# Autodesk Inventor assembly: 膝_6_1
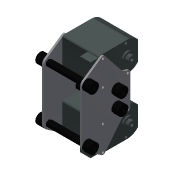
[picture p0: Inventor's stored thumbnail of the model, 180x180]
Saved by Autodesk Inventor 2016 (Build 200138000, 138)
## iProperties
Created: 2016-08-23
Part Number: 膝_6_1
Material: 一般
Document SubType Name: Assembly
Designer: hiro
Mass: 259.679 g
Surface Area: 513.454 cm^2
Volume: 137.54 cm^3
Density: 1.88802 g/cm^3
Author: hiro
## Documents named in this file (11)
- C:\Users\haya\Desktop\OpenPlatform\下半身_160823\膝\膝_6_1_MIR.iam
- C:\Users\haya\Desktop\OpenPlatform\既製品\B3M11xx.ipt
- B3M11xx.ipt
- C:\Users\haya\Desktop\OpenPlatform\下半身_160823\膝\膝_メインフレーム_6_1.ipt
- C:\Users\haya\Desktop\OpenPlatform\下半身_160823\膝\膝_サブフレーム_6_4.ipt
- C:\Users\haya\Desktop\OpenPlatform\既製品\新規購入\AMP-340E.ipt
- C:\Users\haya\Desktop\OpenPlatform\既製品\新規購入\BRU-306_5.ipt
- C:\Users\haya\Desktop\OpenPlatform\既製品\新規購入\D3040-7815B.ipt
- C:\Users\haya\Desktop\OpenPlatform\既製品\新規購入\D3040-7115B.ipt
- C:\Users\haya\Desktop\OpenPlatform\既製品\新規購入\LL-7211-08.ipt
- C:\Users\haya\Desktop\OpenPlatform\既製品\新規購入\LL-7211-10.ipt
## Components (40 placed, 9 different names)
1. B3M11xx:1 — メイト:1, メイト:2, フラッシュ:1, 挿入:1, 挿入:2, 挿入:3, 挿入:7, 挿入:10, 挿入:11
2. 膝_メインフレーム_6_1:1 — 挿入:1, 挿入:2, 挿入:3, 挿入:4, 挿入:5, 挿入:6, 挿入:34, 挿入:35, 挿入:36, 挿入:37, 挿入:38, 挿入:39, 角度:1, 角度:2, 角度:3, 角度:4, 挿入:44, 挿入:45, 挿入:58, 挿入:59, 挿入:60, 挿入:61
3. B3M11xx:2 — 挿入:4, 挿入:5, 挿入:6, 挿入:8, 挿入:9, 挿入:12
4. 膝_メインフレーム_6_1:2 — 挿入:7, 挿入:8, 挿入:9, 挿入:10, 挿入:11, 挿入:12, 挿入:40, 挿入:41, 挿入:42, 挿入:43, メイト:3, メイト:4, メイト:5, メイト:6, メイト:7, メイト:8, メイト:9, メイト:10
5. 膝_サブフレーム_6_4:1 — 挿入:34
6. 膝_サブフレーム_6_4:2 — 挿入:35
7. AMP-340E:1 — 挿入:36, 挿入:43, 角度:1
8. AMP-340E:2 — 挿入:37, 挿入:42, 角度:4
9. AMP-340E:3 — 挿入:38, 挿入:40, 角度:2
10. AMP-340E:4 — 挿入:39, 挿入:41, 角度:3
11. 膝_サブフレーム_6_4:3 — メイト:6, メイト:9, 挿入:56
12. 膝_サブフレーム_6_4:4 — メイト:5, メイト:10, 挿入:54
13. 膝_サブフレーム_6_4:5 — メイト:3, メイト:4, 挿入:55
14. 膝_サブフレーム_6_4:6 — メイト:7, メイト:8, 挿入:57
15. 膝_サブフレーム_6_4:7 — 挿入:44
16. 膝_サブフレーム_6_4:8 — 挿入:45
17. BRU-306_5:1 — 挿入:60, 挿入:93
18. BRU-306_5:2 — 挿入:61, 挿入:92
19. BRU-306_5:3 — 挿入:57, 挿入:90
20. BRU-306_5:4 — 挿入:54, 挿入:88
21. BRU-306_5:5 — 挿入:59, 挿入:91
22. BRU-306_5:6 — 挿入:58, 挿入:87
23. BRU-306_5:7 — 挿入:56, 挿入:89
24. BRU-306_5:8 — 挿入:55, 挿入:86
25. D3040-7815B:1 — 挿入:79, 挿入:90
26. D3040-7815B:2 — 挿入:80, 挿入:88
27. D3040-7815B:3 — 挿入:78, 挿入:86
28. D3040-7815B:4 — 挿入:81, 挿入:89
29. D3040-7115B:1 — 挿入:85, 挿入:91
30. D3040-7115B:2 — 挿入:84, 挿入:92
31. D3040-7115B:3 — 挿入:83, 挿入:93
32. D3040-7115B:4 — 挿入:82, 挿入:87
33. LL-7211-08:1 — 挿入:81
34. LL-7211-08:2 — 挿入:79
35. LL-7211-08:3 — 挿入:80
36. LL-7211-08:4 — 挿入:78
37. LL-7211-10:1 — 挿入:85
38. LL-7211-10:2 — 挿入:82
39. LL-7211-10:3 — 挿入:83
40. LL-7211-10:4 — 挿入:84
## Relationships (63: Insert 48, Mate 10, Angle 4, Flush 1)
- メイト:1 [Mate] (-19.75 mm): B3M11xx:1
- メイト:2 [Mate] (-25.75 mm): B3M11xx:1
- フラッシュ:1 [Flush] (38 mm): B3M11xx:1
- 挿入:1 [Insert]: B3M11xx:1 ↔ 膝_メインフレーム_6_1:1
- 挿入:2 [Insert]: B3M11xx:1 ↔ 膝_メインフレーム_6_1:1
- 挿入:3 [Insert]: B3M11xx:1 ↔ 膝_メインフレーム_6_1:1
- 挿入:4 [Insert]: 膝_メインフレーム_6_1:1 ↔ B3M11xx:2
- 挿入:5 [Insert]: 膝_メインフレーム_6_1:1 ↔ B3M11xx:2
- 挿入:6 [Insert]: 膝_メインフレーム_6_1:1 ↔ B3M11xx:2
- 挿入:7 [Insert]: B3M11xx:1 ↔ 膝_メインフレーム_6_1:2
- 挿入:8 [Insert]: B3M11xx:2 ↔ 膝_メインフレーム_6_1:2
- 挿入:9 [Insert]: B3M11xx:2 ↔ 膝_メインフレーム_6_1:2
- 挿入:10 [Insert]: B3M11xx:1 ↔ 膝_メインフレーム_6_1:2
- 挿入:11 [Insert]: B3M11xx:1 ↔ 膝_メインフレーム_6_1:2
- 挿入:12 [Insert]: B3M11xx:2 ↔ 膝_メインフレーム_6_1:2
- 挿入:34 [Insert]: 膝_メインフレーム_6_1:1 ↔ 膝_サブフレーム_6_4:1
- 挿入:35 [Insert]: 膝_メインフレーム_6_1:1 ↔ 膝_サブフレーム_6_4:2
- 挿入:36 [Insert]: 膝_メインフレーム_6_1:1 ↔ AMP-340E:1
- 挿入:37 [Insert]: 膝_メインフレーム_6_1:1 ↔ AMP-340E:2
- 挿入:38 [Insert]: 膝_メインフレーム_6_1:1 ↔ AMP-340E:3
- 挿入:39 [Insert]: 膝_メインフレーム_6_1:1 ↔ AMP-340E:4
- 挿入:40 [Insert]: 膝_メインフレーム_6_1:2 ↔ AMP-340E:3
- 挿入:41 [Insert]: 膝_メインフレーム_6_1:2 ↔ AMP-340E:4
- 挿入:42 [Insert]: 膝_メインフレーム_6_1:2 ↔ AMP-340E:2
- 挿入:43 [Insert]: 膝_メインフレーム_6_1:2 ↔ AMP-340E:1
- 角度:1 [Angle] (0 deg): 膝_メインフレーム_6_1:1 ↔ AMP-340E:1
- 角度:2 [Angle] (0 deg): 膝_メインフレーム_6_1:1 ↔ AMP-340E:3
- 角度:3 [Angle] (0 deg): 膝_メインフレーム_6_1:1 ↔ AMP-340E:4
- 角度:4 [Angle] (0 deg): 膝_メインフレーム_6_1:1 ↔ AMP-340E:2
- メイト:3 [Mate]: 膝_メインフレーム_6_1:2 ↔ 膝_サブフレーム_6_4:5
- メイト:4 [Mate]: 膝_メインフレーム_6_1:2 ↔ 膝_サブフレーム_6_4:5
- メイト:5 [Mate]: 膝_メインフレーム_6_1:2 ↔ 膝_サブフレーム_6_4:4
- メイト:6 [Mate]: 膝_メインフレーム_6_1:2 ↔ 膝_サブフレーム_6_4:3
- メイト:7 [Mate]: 膝_メインフレーム_6_1:2 ↔ 膝_サブフレーム_6_4:6
- メイト:8 [Mate]: 膝_メインフレーム_6_1:2 ↔ 膝_サブフレーム_6_4:6
- メイト:9 [Mate]: 膝_メインフレーム_6_1:2 ↔ 膝_サブフレーム_6_4:3
- メイト:10 [Mate]: 膝_メインフレーム_6_1:2 ↔ 膝_サブフレーム_6_4:4
- 挿入:44 [Insert]: 膝_メインフレーム_6_1:1 ↔ 膝_サブフレーム_6_4:7
- 挿入:45 [Insert]: 膝_メインフレーム_6_1:1 ↔ 膝_サブフレーム_6_4:8
- 挿入:54 [Insert]: 膝_サブフレーム_6_4:4 ↔ BRU-306_5:4
- 挿入:55 [Insert]: 膝_サブフレーム_6_4:5 ↔ BRU-306_5:8
- 挿入:56 [Insert]: 膝_サブフレーム_6_4:3 ↔ BRU-306_5:7
- 挿入:57 [Insert]: 膝_サブフレーム_6_4:6 ↔ BRU-306_5:3
- 挿入:58 [Insert]: 膝_メインフレーム_6_1:1 ↔ BRU-306_5:6
- 挿入:59 [Insert]: 膝_メインフレーム_6_1:1 ↔ BRU-306_5:5
- 挿入:60 [Insert]: 膝_メインフレーム_6_1:1 ↔ BRU-306_5:1
- 挿入:61 [Insert]: 膝_メインフレーム_6_1:1 ↔ BRU-306_5:2
- 挿入:78 [Insert]: D3040-7815B:3 ↔ LL-7211-08:4
- 挿入:79 [Insert]: D3040-7815B:1 ↔ LL-7211-08:2
- 挿入:80 [Insert]: D3040-7815B:2 ↔ LL-7211-08:3
- 挿入:81 [Insert]: D3040-7815B:4 ↔ LL-7211-08:1
- 挿入:82 [Insert]: D3040-7115B:4 ↔ LL-7211-10:2
- 挿入:83 [Insert]: D3040-7115B:3 ↔ LL-7211-10:3
- 挿入:84 [Insert]: D3040-7115B:2 ↔ LL-7211-10:4
- 挿入:85 [Insert]: D3040-7115B:1 ↔ LL-7211-10:1
- 挿入:86 [Insert]: BRU-306_5:8 ↔ D3040-7815B:3
- 挿入:87 [Insert]: BRU-306_5:6 ↔ D3040-7115B:4
- 挿入:88 [Insert]: BRU-306_5:4 ↔ D3040-7815B:2
- 挿入:89 [Insert]: BRU-306_5:7 ↔ D3040-7815B:4
- 挿入:90 [Insert]: BRU-306_5:3 ↔ D3040-7815B:1
- 挿入:91 [Insert]: BRU-306_5:5 ↔ D3040-7115B:1
- 挿入:92 [Insert]: BRU-306_5:2 ↔ D3040-7115B:2
- 挿入:93 [Insert]: BRU-306_5:1 ↔ D3040-7115B:3
## Named parameters: sa_0 = 0, sa_1 = 800000, sa_2 = 0
note: some values were not read from the file. Shown as the stored number, unit unknown: "sa_0", "sa_1", "sa_2".
